# Autodesk Inventor assembly: Cable Tie Assembly
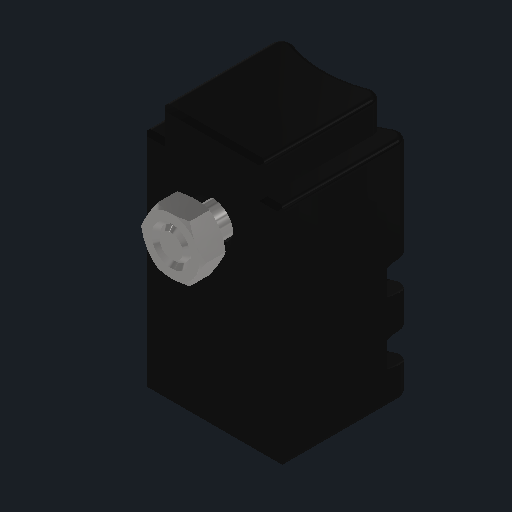
[picture p0: Inventor's stored thumbnail of the model, 512x512]
Saved by Autodesk Inventor 2025.1 (Build 291241020, 241B)
## iProperties
Created: 2025-05-11
Part Number: Cable Tie Assembly
Document SubType Name: Assembly
Designer: Joshua Eah
Author: Joshua Eah
## Documents named in this file (4)
- C:\Users\Joshua Eah\Documents\Voron 0.2\CAD\Master Assembly\Cable Tie Assembly.iam
- C:\Users\Joshua Eah\Documents\Voron 0.2\CAD\Master Assembly\Cable Tie.ipt
- C:\Users\Joshua Eah\Documents\Voron 0.2\CAD\Master Assembly\Hardware\M3x10 BHCS.ipt
- C:\Users\Joshua Eah\Documents\Voron 0.2\CAD\Master Assembly\Hardware\M3 Hexnut.ipt
## Components (3 placed, 3 different names)
1. Cable Tie:1
2. M3x10 BHCS:1
3. M3 Hexnut:9
## Relationships (2: Insert 2)
- [Insert]: M3x10 BHCS:1 ↔ M3 Hexnut:9
- [Insert]: Cable Tie:1 ↔ M3x10 BHCS:1
